# Autodesk Inventor assembly: 68072RS
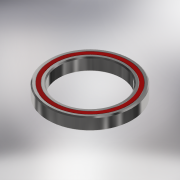
[picture p0: Inventor's stored thumbnail of the model, 180x180]
Saved by Autodesk Inventor 2017 (Build 210142000, 142)
## iProperties
Created: 2016-08-26
Part Number: 68072RS
Document SubType Name: Assembly
Designer: Ali
Author: Ali
## Documents named in this file (3)
- C:\Users\Ali\Dropbox\Work\Project\Inventor\Parts\68072RS.iam
- C:\Users\Ali\Dropbox\Work\Project\Inventor\Parts\6807-outer.ipt
- C:\Users\Ali\Dropbox\Work\Project\Inventor\Parts\6807-inner.ipt
## Components (2 placed, 2 different names)
1. 6807-outer:1 — Rotational:1
2. 6807-inner:1 — Rotational:1
## Relationships (1: RevoluteJoint 1)
- Rotational:1 [RevoluteJoint]: 6807-outer:1 ↔ 6807-inner:1
